# Autodesk Inventor assembly: Elevator
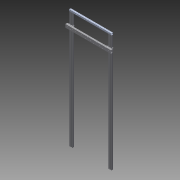
[picture p0: Inventor's stored thumbnail of the model, 180x180]
Saved by Autodesk Inventor 2015 (Build 190159000, 159)
## iProperties
Created: 2015-01-25
Part Number: Elevator
Document SubType Name: Assembly
Designer: cstewart1
Author: cstewart1
## Documents named in this file (4)
- C:\Users\cstewart1\Inventor\HWRobot2015CAD\Elevator\Elevator.iam
- C:\Users\cstewart1\Inventor\HWRobot2015CAD\FRCKOP2015\McMaster\47065T125.ipt
- C:\Users\cstewart1\Inventor\HWRobot2015CAD\FRCKOP2015\VersaFrame\217-3426-STEP.ipt
- C:\Users\cstewart1\Inventor\HWRobot2015CAD\Elevator\ForkLift.iam
## Components (4 placed, 3 different names)
1. 47065T125:1 — Flush:1, Flush:2, Flush:5, Flush:6, Slider:1
2. ForkCar [sub-assembly] — Slider:1, Mate:1
3. 47065T125:2 — Flush:1, Flush:2, Flush:5, Mate:1
4. 217-3426-STEP:1 — Flush:6
## Relationships (6: Flush 4, TranslationJoint 1, Mate 1)
- Flush:1: 47065T125:1 ↔ 47065T125:2
- Flush:2: 47065T125:1 ↔ 47065T125:2
- Flush:5: 47065T125:1 ↔ 47065T125:2
- Flush:6: 47065T125:1 ↔ 217-3426-STEP:1
- Slider:1 [TranslationJoint] (6.35 mm): 47065T125:1 ↔ ForkCar
- Mate:1 (5.842 mm): ForkCar ↔ 47065T125:2
